# Autodesk Inventor assembly: ARM_013_RollerBar
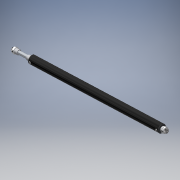
[picture p0: Inventor's stored thumbnail of the model, 180x180]
Saved by Autodesk Inventor 2018.3 (Build 223284000, 284)
## iProperties
Created: 2020-02-02
Part Number: ARM_013_RollerBar
Document SubType Name: Assembly
Designer: 22barlalex
Mass: 397.432 g
Surface Area: 2208.83 cm^2
Volume: 265.41 cm^3
Density: 1.49743 g/cm^3
Author: 22barlalex
## Documents named in this file (12)
- C:\Users\22barlalex\Documents\GrabCAD\Infinite Recharge 2020\Build season\ARM_013_RollerBar.iam
- C:\Users\22barlalex\Documents\GrabCAD\Infinite Recharge 2020\Build season\ARM_015_VersaRoller_Hub_1_2_Hex_Bore_x_1-1_8_OD_Aluminum_217-5895.ipt
- C:\Users\22barlalex\Documents\GrabCAD\Infinite Recharge 2020\Build season\ARM_016_VersaRoller_Tube_1-_OD_x_1-_ID_x_1_16_Wall_Aluminum_59_217-5901.ipt
- C:\Users\22barlalex\Documents\GrabCAD\Infinite Recharge 2020\Build season\ARM_017_VersaRoller_1_2_Hex_Hub_Insert_1_2_Hex_Shaft_x_2-1_2_Long_217-5899.ipt
- C:\Users\22barlalex\Documents\GrabCAD\Infinite Recharge 2020\Build season\ARM_019_0_375_ID_x_0_875_OD_x_0_280_WD_Flanged_Bearing_217-2733.ipt
- C:\Users\22barlalex\Documents\GrabCAD\Infinite Recharge 2020\Build season\ARM_021_91259A176_ALLOY STEEL SHOULDER SCREW.ipt
- C:\Users\22barlalex\Documents\GrabCAD\Infinite Recharge 2020\Build season\ARM_022_5234K910_SUPER SOFT LATEX RUBBER TUBING.ipt
- C:\Users\22barlalex\Documents\GrabCAD\Infinite Recharge 2020\Build season\ARM_018_0.5inHexSpacer.ipt
- C:\Users\22barlalex\Documents\GrabCAD\Infinite Recharge 2020\Build season\ARM_025_VersaRoller_1_2_Hex_Hub_Insert_5_16-18_Tapped_Hole_217-5897.ipt
- C:\Users\22barlalex\Documents\GrabCAD\Infinite Recharge 2020\Build season\ARM_026_.25inHexSpacer.ipt
- C:\Users\22barlalex\Documents\GrabCAD\Infinite Recharge 2020\Build season\ARM_028_ANSI B18.3 - 10-24 UNC - UNC - 0.1875.ipt
- C:\Users\22barlalex\Documents\GrabCAD\Infinite Recharge 2020\Build season\ARM_027_ANSI B18.3 - 5_16-18 UNC - UNC - 0.5.ipt
## Components (18 placed, 11 different names)
1. ARM_015_VersaRoller_Hub_1_2_Hex_Bore_x_1-1_8_OD_Aluminum_217-5895:1 — Mate:13, Mate:41, Flush:1, Mate:59
2. ARM_016_VersaRoller_Tube_1-_OD_x_1-_ID_x_1_16_Wall_Aluminum_59_217-5901:1 — Mate:7, Mate:13, Mate:18, Mate:25, Mate:48, Mate:49, Mate:50, Mate:51, Mate:52, Mate:53, Mate:54, Mate:55, Mate:60
3. ARM_017_VersaRoller_1_2_Hex_Hub_Insert_1_2_Hex_Shaft_x_2-1_2_Long_217-5899:1 — Mate:18, Mate:24, Mate:33, Mate:36, Mate:38, Insert:1, Mate:62, Mate:63
4. ARM_015_VersaRoller_Hub_1_2_Hex_Bore_x_1-1_8_OD_Aluminum_217-5895:2 — Mate:7, Mate:57, Mate:58
5. ARM_019_0_375_ID_x_0_875_OD_x_0_280_WD_Flanged_Bearing_217-2733:1 — Mate:22, Mate:23, Mate:24, Mate:39
6. ARM_019_0_375_ID_x_0_875_OD_x_0_280_WD_Flanged_Bearing_217-2733:2 — Mate:20, Mate:21, Mate:47
7. ARM_021_91259A176_ALLOY STEEL SHOULDER SCREW:1 — Mate:20, Mate:21, Mate:44
8. ARM_021_91259A176_ALLOY STEEL SHOULDER SCREW:2 — Mate:22, Mate:23, Mate:63
9. ARM_022_5234K910_SUPER SOFT LATEX RUBBER TUBING:1 — Mate:25, Mate:56
10. ARM_018_0.5inHexSpacer:1 — Mate:33, Mate:39, Mate:61, Mate:62
11. ARM_018_0.5inHexSpacer:2 — Mate:36, Mate:38, Mate:61
12. ARM_025_VersaRoller_1_2_Hex_Hub_Insert_5_16-18_Tapped_Hole_217-5897:1 — Mate:41, Mate:44, Mate:45, Mate:46, Flush:1
13. ARM_026_.25inHexSpacer:1 — Mate:45, Mate:46, Mate:47
14. Hexagon Socket Button Head Cap Screw - Inch 10 - 24 x 3/16:1 — Mate:52, Mate:53
15. Hexagon Socket Button Head Cap Screw - Inch 10 - 24 x 3/16:2 — Mate:54, Mate:55, Mate:56, Mate:59, Mate:60
16. Hexagon Socket Button Head Cap Screw - Inch 10 - 24 x 3/16:3 — Mate:48, Mate:49, Mate:58
17. Hexagon Socket Button Head Cap Screw - Inch 10 - 24 x 3/16:4 — Mate:50, Mate:51
18. Hexagon Socket Button Head Cap Screw - Inch 5/16 - 18 x 1/2:2 — Insert:1, Mate:57
## Relationships (36: Mate 34, Insert 1, Flush 1)
- Mate:7: ARM_016_VersaRoller_Tube_1-_OD_x_1-_ID_x_1_16_Wall_Aluminum_59_217-5901:1 ↔ ARM_015_VersaRoller_Hub_1_2_Hex_Bore_x_1-1_8_OD_Aluminum_217-5895:2
- Mate:13: ARM_015_VersaRoller_Hub_1_2_Hex_Bore_x_1-1_8_OD_Aluminum_217-5895:1 ↔ ARM_016_VersaRoller_Tube_1-_OD_x_1-_ID_x_1_16_Wall_Aluminum_59_217-5901:1
- Mate:18: ARM_016_VersaRoller_Tube_1-_OD_x_1-_ID_x_1_16_Wall_Aluminum_59_217-5901:1 ↔ ARM_017_VersaRoller_1_2_Hex_Hub_Insert_1_2_Hex_Shaft_x_2-1_2_Long_217-5899:1
- Mate:20: ARM_019_0_375_ID_x_0_875_OD_x_0_280_WD_Flanged_Bearing_217-2733:2 ↔ ARM_021_91259A176_ALLOY STEEL SHOULDER SCREW:1
- Mate:21: ARM_019_0_375_ID_x_0_875_OD_x_0_280_WD_Flanged_Bearing_217-2733:2 ↔ ARM_021_91259A176_ALLOY STEEL SHOULDER SCREW:1
- Mate:22: ARM_019_0_375_ID_x_0_875_OD_x_0_280_WD_Flanged_Bearing_217-2733:1 ↔ ARM_021_91259A176_ALLOY STEEL SHOULDER SCREW:2
- Mate:23: ARM_019_0_375_ID_x_0_875_OD_x_0_280_WD_Flanged_Bearing_217-2733:1 ↔ ARM_021_91259A176_ALLOY STEEL SHOULDER SCREW:2
- Mate:24: ARM_017_VersaRoller_1_2_Hex_Hub_Insert_1_2_Hex_Shaft_x_2-1_2_Long_217-5899:1 ↔ ARM_019_0_375_ID_x_0_875_OD_x_0_280_WD_Flanged_Bearing_217-2733:1
- Mate:25: ARM_016_VersaRoller_Tube_1-_OD_x_1-_ID_x_1_16_Wall_Aluminum_59_217-5901:1 ↔ ARM_022_5234K910_SUPER SOFT LATEX RUBBER TUBING:1
- Mate:33: ARM_017_VersaRoller_1_2_Hex_Hub_Insert_1_2_Hex_Shaft_x_2-1_2_Long_217-5899:1 ↔ ARM_018_0.5inHexSpacer:1
- Mate:36: ARM_017_VersaRoller_1_2_Hex_Hub_Insert_1_2_Hex_Shaft_x_2-1_2_Long_217-5899:1 ↔ ARM_018_0.5inHexSpacer:2
- Mate:38: ARM_017_VersaRoller_1_2_Hex_Hub_Insert_1_2_Hex_Shaft_x_2-1_2_Long_217-5899:1 ↔ ARM_018_0.5inHexSpacer:2
- Mate:39: ARM_019_0_375_ID_x_0_875_OD_x_0_280_WD_Flanged_Bearing_217-2733:1 ↔ ARM_018_0.5inHexSpacer:1
- Mate:41: ARM_015_VersaRoller_Hub_1_2_Hex_Bore_x_1-1_8_OD_Aluminum_217-5895:1 ↔ ARM_025_VersaRoller_1_2_Hex_Hub_Insert_5_16-18_Tapped_Hole_217-5897:1
- Mate:44: ARM_021_91259A176_ALLOY STEEL SHOULDER SCREW:1 ↔ ARM_025_VersaRoller_1_2_Hex_Hub_Insert_5_16-18_Tapped_Hole_217-5897:1
- Mate:45: ARM_025_VersaRoller_1_2_Hex_Hub_Insert_5_16-18_Tapped_Hole_217-5897:1 ↔ ARM_026_.25inHexSpacer:1
- Mate:46: ARM_025_VersaRoller_1_2_Hex_Hub_Insert_5_16-18_Tapped_Hole_217-5897:1 ↔ ARM_026_.25inHexSpacer:1
- Mate:47: ARM_019_0_375_ID_x_0_875_OD_x_0_280_WD_Flanged_Bearing_217-2733:2 ↔ ARM_026_.25inHexSpacer:1
- Mate:48: ARM_016_VersaRoller_Tube_1-_OD_x_1-_ID_x_1_16_Wall_Aluminum_59_217-5901:1 ↔ Hexagon Socket Button Head Cap Screw - Inch 10 - 24 x 3/16:3
- Mate:49: ARM_016_VersaRoller_Tube_1-_OD_x_1-_ID_x_1_16_Wall_Aluminum_59_217-5901:1 ↔ Hexagon Socket Button Head Cap Screw - Inch 10 - 24 x 3/16:3
- Mate:50: ARM_016_VersaRoller_Tube_1-_OD_x_1-_ID_x_1_16_Wall_Aluminum_59_217-5901:1 ↔ Hexagon Socket Button Head Cap Screw - Inch 10 - 24 x 3/16:4
- Mate:51: ARM_016_VersaRoller_Tube_1-_OD_x_1-_ID_x_1_16_Wall_Aluminum_59_217-5901:1 ↔ Hexagon Socket Button Head Cap Screw - Inch 10 - 24 x 3/16:4
- Mate:52: ARM_016_VersaRoller_Tube_1-_OD_x_1-_ID_x_1_16_Wall_Aluminum_59_217-5901:1 ↔ Hexagon Socket Button Head Cap Screw - Inch 10 - 24 x 3/16:1
- Mate:53: ARM_016_VersaRoller_Tube_1-_OD_x_1-_ID_x_1_16_Wall_Aluminum_59_217-5901:1 ↔ Hexagon Socket Button Head Cap Screw - Inch 10 - 24 x 3/16:1
- Mate:54: ARM_016_VersaRoller_Tube_1-_OD_x_1-_ID_x_1_16_Wall_Aluminum_59_217-5901:1 ↔ Hexagon Socket Button Head Cap Screw - Inch 10 - 24 x 3/16:2
- Mate:55: ARM_016_VersaRoller_Tube_1-_OD_x_1-_ID_x_1_16_Wall_Aluminum_59_217-5901:1 ↔ Hexagon Socket Button Head Cap Screw - Inch 10 - 24 x 3/16:2
- Mate:56 (6.35 mm): ARM_022_5234K910_SUPER SOFT LATEX RUBBER TUBING:1 ↔ Hexagon Socket Button Head Cap Screw - Inch 10 - 24 x 3/16:2
- Insert:1: ARM_017_VersaRoller_1_2_Hex_Hub_Insert_1_2_Hex_Shaft_x_2-1_2_Long_217-5899:1 ↔ Hexagon Socket Button Head Cap Screw - Inch 5/16 - 18 x 1/2:2
- Mate:57: ARM_015_VersaRoller_Hub_1_2_Hex_Bore_x_1-1_8_OD_Aluminum_217-5895:2 ↔ Hexagon Socket Button Head Cap Screw - Inch 5/16 - 18 x 1/2:2
- Mate:58: ARM_015_VersaRoller_Hub_1_2_Hex_Bore_x_1-1_8_OD_Aluminum_217-5895:2 ↔ Hexagon Socket Button Head Cap Screw - Inch 10 - 24 x 3/16:3
- Flush:1: ARM_015_VersaRoller_Hub_1_2_Hex_Bore_x_1-1_8_OD_Aluminum_217-5895:1 ↔ ARM_025_VersaRoller_1_2_Hex_Hub_Insert_5_16-18_Tapped_Hole_217-5897:1
- Mate:59: ARM_015_VersaRoller_Hub_1_2_Hex_Bore_x_1-1_8_OD_Aluminum_217-5895:1 ↔ Hexagon Socket Button Head Cap Screw - Inch 10 - 24 x 3/16:2
- Mate:60: ARM_016_VersaRoller_Tube_1-_OD_x_1-_ID_x_1_16_Wall_Aluminum_59_217-5901:1 ↔ Hexagon Socket Button Head Cap Screw - Inch 10 - 24 x 3/16:2
- Mate:61: ARM_018_0.5inHexSpacer:1 ↔ ARM_018_0.5inHexSpacer:2
- Mate:62: ARM_017_VersaRoller_1_2_Hex_Hub_Insert_1_2_Hex_Shaft_x_2-1_2_Long_217-5899:1 ↔ ARM_018_0.5inHexSpacer:1
- Mate:63: ARM_017_VersaRoller_1_2_Hex_Hub_Insert_1_2_Hex_Shaft_x_2-1_2_Long_217-5899:1 ↔ ARM_021_91259A176_ALLOY STEEL SHOULDER SCREW:2
